# Autodesk Inventor assembly: aluminium engine v2
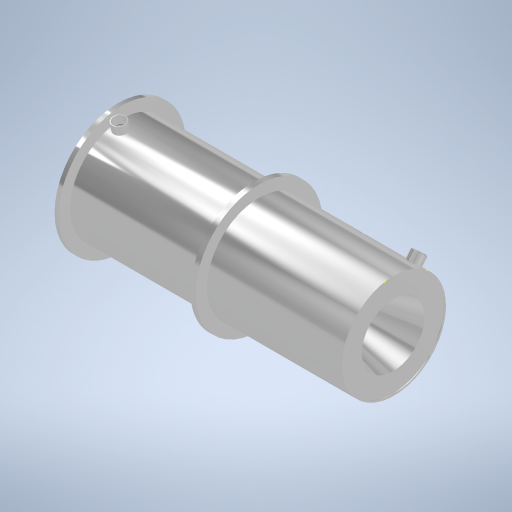
[picture p0: Inventor's stored thumbnail of the model, 512x512]
Saved by Autodesk Inventor 2023 (Build 270158000, 158)
## iProperties
Created: 2022-09-29
Part Number: aluminium engine v2
Document SubType Name: Assembly
Designer: station
Author: station
## Documents named in this file (5)
- C:\Users\station\Documents\Project\Liquid-engine-cooling-system\design files\ethanol engine 6\Aluminium engine v2\aluminium engine v2.iam
- C:\Users\station\Documents\Project\Liquid-engine-cooling-system\design files\ethanol engine 6\Aluminium engine v2\aluminium engine v2.ipt
- C:\Users\station\Documents\Project\Liquid-engine-cooling-system\design files\ethanol engine 6\Aluminium engine v2\stainless steel space.ipt
- C:\Users\station\Documents\Project\Liquid-engine-cooling-system\design files\ethanol engine 6\Aluminium engine v2\aluminium outer wall - front.ipt
- C:\Users\station\Documents\Project\Liquid-engine-cooling-system\design files\ethanol engine 6\Aluminium engine v2\aluminium outer wall back.ipt
## Components (4 placed, 4 different names)
1. aluminium engine v2:1 — Mate:1, Mate:2, Mate:6, Mate:7
2. stainless steel space:1 — Mate:1, Mate:2, Mate:5
3. aluminium outer wall - front:1 — Mate:6, Mate:7, Mate:8
4. aluminium outer wall back:1 — Mate:5, Mate:8
## Relationships (6: Mate 6)
- Mate:1: aluminium engine v2:1 ↔ stainless steel space:1
- Mate:2 (13.716 mm): aluminium engine v2:1 ↔ stainless steel space:1
- Mate:5: stainless steel space:1 ↔ aluminium outer wall back:1
- Mate:6: aluminium engine v2:1 ↔ aluminium outer wall - front:1
- Mate:7: aluminium engine v2:1 ↔ aluminium outer wall - front:1
- Mate:8: aluminium outer wall - front:1 ↔ aluminium outer wall back:1
